# Autodesk Inventor assembly: SAR330
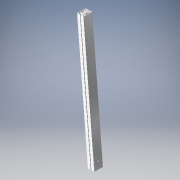
[picture p0: Inventor's stored thumbnail of the model, 180x180]
Saved by Autodesk Inventor 2019 (Build 230136000, 136)
## iProperties
Category: PARTsolutions
Company: MISUMI
Created: 2019-04-19
Part Number: SAR330
Catalog Web Link: www.cadenas.de
Description: SAR3-Slide Rails - Aluminum Alloy - Three-Step Slide Rails
Vendor: MISUMI
Document SubType Name: Assembly
Designer: psadmin
Manufacturer: MISUMI
Mass: 180.874 g
Surface Area: 598.523 cm^2
Volume: 66.9905 cm^3
Density: 2.7 g/cm^3
Title: SAR330
Author: Cadenas PARTsolutions
Comments: Slide Rails - Aluminum Alloy - Three-Step Slide Rails
## Documents named in this file (4)
- C:\Robotics\CAD\COTSParts\Misumi_Slides\AIS2018\SAR330.iam
- C:\Robotics\CAD\COTSParts\Misumi_Slides\AIS2018\SAR330-30_r.ipt
- C:\Robotics\CAD\COTSParts\Misumi_Slides\AIS2018\SAR330-30_b.ipt
- C:\Robotics\CAD\COTSParts\Misumi_Slides\AIS2018\ball bearing replacement.ipt
## Components (7 placed, 3 different names)
1. SAR330-30_r:1 — Flush:2, Mate:3, Mate:4, Mate:7, Mate:8, Flush:3, Mate:10
2. SAR330-30_b:1 — Flush:1, Flush:2, Mate:1, Mate:2, Flush:3, Flush:4
3. SAR330-30_b:2 — Flush:1, Mate:5, Mate:6, Mate:9, Mate:10, Flush:4
4. ball bearing replacement:1 — Mate:2, Mate:4
5. ball bearing replacement:2 — Mate:1, Mate:3
6. ball bearing replacement:3 — Mate:5, Mate:8
7. ball bearing replacement:4 — Mate:6, Mate:7, Mate:9
## Relationships (14: Mate 10, Flush 4)
- Flush:1: SAR330-30_b:1 ↔ SAR330-30_b:2
- Flush:2: SAR330-30_r:1 ↔ SAR330-30_b:1
- Mate:1: SAR330-30_b:1 ↔ ball bearing replacement:2
- Mate:2: SAR330-30_b:1 ↔ ball bearing replacement:1
- Mate:3: SAR330-30_r:1 ↔ ball bearing replacement:2
- Mate:4: SAR330-30_r:1 ↔ ball bearing replacement:1
- Mate:5: SAR330-30_b:2 ↔ ball bearing replacement:3
- Mate:6: SAR330-30_b:2 ↔ ball bearing replacement:4
- Mate:7: SAR330-30_r:1 ↔ ball bearing replacement:4
- Mate:8: SAR330-30_r:1 ↔ ball bearing replacement:3
- Mate:9 (-6.35 mm): SAR330-30_b:2 ↔ ball bearing replacement:4
- Flush:3: SAR330-30_r:1 ↔ SAR330-30_b:1
- Mate:10 (-25.4 mm): SAR330-30_r:1 ↔ SAR330-30_b:2
- Flush:4: SAR330-30_b:1 ↔ SAR330-30_b:2
